# Autodesk Inventor assembly: Head
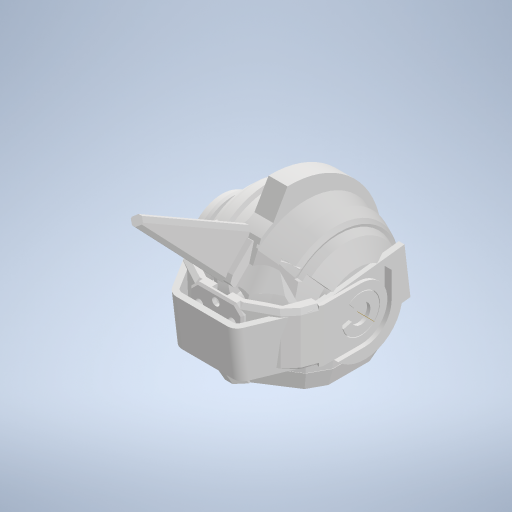
[picture p0: Inventor's stored thumbnail of the model, 512x512]
Saved by Autodesk Inventor 2024.1 (Build 281209000, 209)
## iProperties
Created: 2024-02-18
Part Number: Head
Document SubType Name: Assembly
Designer: hibik
Author: hibik
## Documents named in this file (11)
- C:\Users\hibik\Desktop\ロボメカ\HR\2024.02.11 Rl\02.11 ProtType\Head.iam
- C:\Users\hibik\Desktop\ロボメカ\HR\2024.02.11 Rl\02.11 ProtType\Head_2.ipt
- C:\Users\hibik\Desktop\ロボメカ\HR\2024.02.11 Rl\02.11 ProtType\Head_1.ipt
- C:\Users\hibik\Desktop\ロボメカ\HR\2024.02.11 Rl\02.11 ProtType\Head_3.ipt
- C:\Users\hibik\Desktop\ロボメカ\HR\2024.02.11 Rl\02.11 ProtType\Head_4.ipt
- C:\Users\hibik\Desktop\ロボメカ\HR\2024.02.11 Rl\02.11 ProtType\Head_cover.ipt
- C:\Users\hibik\Desktop\ロボメカ\HR\2024.02.11 Rl\02.11 ProtType\Head_eye.ipt
- C:\Users\hibik\Desktop\ロボメカ\HR\2024.02.11 Rl\02.11 ProtType\Head_year_left.ipt
- C:\Users\hibik\Desktop\ロボメカ\HR\2024.02.11 Rl\02.11 ProtType\Head_year_right.ipt
- C:\Users\hibik\Desktop\ロボメカ\HR\2024.02.11 Rl\KRS3300サーボホーン.ipt
- C:\Users\hibik\Desktop\ロボメカ\HR\2024.02.11 Rl\02.11 ProtType\Head_cover_CNC.ipt
## Components (10 placed, 10 different names)
1. Head_2:1 — メイト:2, メイト:3, メイト:4, 挿入:7
2. Head_1:1 — メイト:2, メイト:3, メイト:4, メイト:5, メイト:6, 挿入:1, 挿入:2
3. Head_3:1 — メイト:6, 挿入:2, 挿入:3
4. Head_4:1 — メイト:5, 挿入:1, 挿入:5, 挿入:6
5. Head_cover:1 — 挿入:6
6. Head_eye:1 — 挿入:3
7. Head_year_left:1
8. Head_year_right:1 — 挿入:5
9. KRS3300サーボホーン:1 — 挿入:7
10. Head_cover_CNC:1
## Relationships (11: Insert 6, Mate 5)
- メイト:2 [Mate]: Head_2:1 ↔ Head_1:1
- メイト:3 [Mate]: Head_2:1 ↔ Head_1:1
- メイト:4 [Mate]: Head_2:1 ↔ Head_1:1
- メイト:5 [Mate]: Head_1:1 ↔ Head_4:1
- メイト:6 [Mate]: Head_1:1 ↔ Head_3:1
- 挿入:1 [Insert]: Head_1:1 ↔ Head_4:1
- 挿入:2 [Insert]: Head_1:1 ↔ Head_3:1
- 挿入:3 [Insert]: Head_3:1 ↔ Head_eye:1
- 挿入:5 [Insert]: Head_4:1 ↔ Head_year_right:1
- 挿入:6 [Insert]: Head_4:1 ↔ Head_cover:1
- 挿入:7 [Insert]: Head_2:1 ↔ KRS3300サーボホーン:1
